# Autodesk Inventor assembly: poot met 2 dwarsprofielen
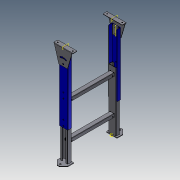
[picture p0: Inventor's stored thumbnail of the model, 180x180]
Saved by Autodesk Inventor 2015 SP1 (Build 190203100, 203)
## iProperties
Created: 2007-07-03
Part Number: poot met 2 dwarsprofielen
Document SubType Name: Assembly
Designer: kurt
Manufacturer: Standard
Standards Organization: Custom
Author: kurt
## Documents named in this file (6)
- F:\Tekeningen\bibliotheek\poten\Sub-assemblys\poot 700-900.iam
- F:\Tekeningen\bibliotheek\poten\Sub-assemblys\90-10-0550.iam
- F:\Tekeningen\bibliotheek\poten\onderdelen\90-04-0580.ipt
- F:\Tekeningen\bibliotheek\poten\onderdelen\90-09-0500.ipt
- F:\Tekeningen\bibliotheek\poten\onderdelen\90-02-0000.ipt
- F:\Tekeningen\bibliotheek\poten\onderdelen\90-03-0000.ipt
## Components (12 placed, 5 different names)
1. 90-04-0580:1 — Insert:4, Insert:5, Insert:6, Insert:7, Insert:12, Flush:11, Mate:31, Mate:33
2. 90-04-0580:2 — Insert:8, Insert:9, Insert:10, Insert:11, Insert:13, Mate:32, Flush:12
3. 90-02-0000:1 — Flush:8, Angle:1, Insert:13
4. 90-02-0000:2 — Flush:8, Insert:12, Angle:1, Mate:33
5. 90-03-0000:1 — Insert:8, Insert:9
6. 90-03-0000:2 — Insert:4, Insert:5
7. 90-03-0000:3 — Insert:6, Insert:7
8. 90-03-0000:4 — Insert:10, Insert:11
9. 90-10-0550:1 [sub-assembly] — Mate:27, Flush:9, Mate:28, Insert:1, Mate:29, Insert:3, Mate:30, Flush:11, Mate:31
10. 90-10-0550:2 [sub-assembly] — Insert:2, Flush:10, Mate:32, Flush:12
11. 90-09-0500:1 — Insert:1, Mate:29, Insert:2, Flush:10
12. 90-09-0500:2 — Insert:3, Mate:30
## Relationships (26: Insert 13, Mate 7, Flush 5, Angle 1)
- Flush:8: 90-02-0000:1 ↔ 90-02-0000:2
- Mate:27: 90-10-0550:1
- Flush:9: 90-10-0550:1
- Mate:28: 90-10-0550:1
- Insert:1 (1 mm): 90-10-0550:1 ↔ 90-09-0500:1
- Mate:29: 90-10-0550:1 ↔ 90-09-0500:1
- Insert:2 (1 mm): 90-10-0550:2 ↔ 90-09-0500:1
- Flush:10: 90-10-0550:2 ↔ 90-09-0500:1
- Insert:3 (1 mm): 90-10-0550:1 ↔ 90-09-0500:2
- Mate:30: 90-10-0550:1 ↔ 90-09-0500:2
- Insert:4 (3 mm): 90-04-0580:1 ↔ 90-03-0000:2
- Insert:5 (3 mm): 90-04-0580:1 ↔ 90-03-0000:2
- Insert:6: 90-04-0580:1 ↔ 90-03-0000:3
- Insert:7: 90-04-0580:1 ↔ 90-03-0000:3
- Insert:8: 90-04-0580:2 ↔ 90-03-0000:1
- Insert:9: 90-04-0580:2 ↔ 90-03-0000:1
- Insert:10 (3 mm): 90-04-0580:2 ↔ 90-03-0000:4
- Insert:11 (3 mm): 90-04-0580:2 ↔ 90-03-0000:4
- Insert:12: 90-04-0580:1 ↔ 90-02-0000:2
- Angle:1 (0 deg): 90-02-0000:1 ↔ 90-02-0000:2
- Insert:13: 90-04-0580:2 ↔ 90-02-0000:1
- Flush:11: 90-04-0580:1 ↔ 90-10-0550:1
- Mate:31: 90-04-0580:1 ↔ 90-10-0550:1
- Mate:32: 90-04-0580:2 ↔ 90-10-0550:2
- Flush:12: 90-04-0580:2 ↔ 90-10-0550:2
- Mate:33: 90-04-0580:1 ↔ 90-02-0000:2
